# Autodesk Inventor assembly: mewa
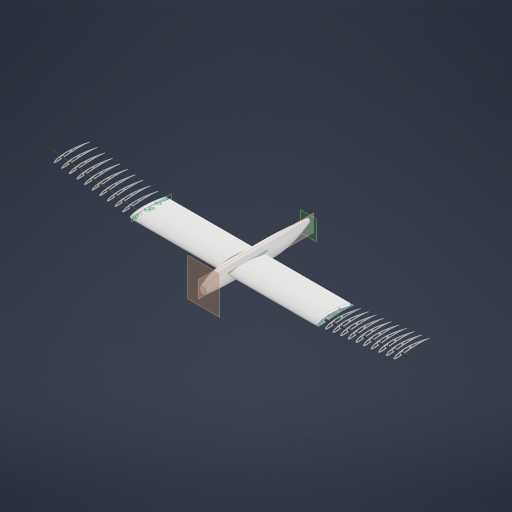
[picture p0: Inventor's stored thumbnail of the model, 512x512]
Saved by Autodesk Inventor 2023 (Build 270158000, 158)
## iProperties
Created: 2022-12-16
Part Number: mewa
Document SubType Name: Assembly
Designer: szykr
Mass: 3067.96 g
Surface Area: 12707.3 cm^2
Volume: 3076.29 cm^3
Density: 0.997294 g/cm^3
Author: szykr
## Documents named in this file (3)
- D:\Folder Instalacyjny\GitHub Pliki\Solaris\model\mewa.iam
- D:\Folder Instalacyjny\GitHub Pliki\Solaris\model\Kadłub v3.ipt
- D:\Folder Instalacyjny\GitHub Pliki\Solaris\model\Skrzydło.iam
## Components (2 placed, 2 different names)
1. Kadłub v3:1 — Rigid:1
2. Skrzydło:1 [sub-assembly] — Rigid:1
## Relationships (1: WeldJoint 1)
- Rigid:1 [WeldJoint] (-35.613 mm): Kadłub v3:1 ↔ Skrzydło:1
